# Autodesk Inventor assembly: поршень_шатун_палец
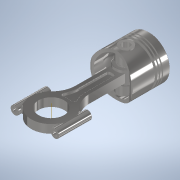
[picture p0: Inventor's stored thumbnail of the model, 180x180]
Saved by Autodesk Inventor 2021 (Build 250183000, 183)
## iProperties
Created: 2021-06-15
Part Number: поршень_шатун_палец
Document SubType Name: Assembly
Designer: panda
Author: panda
## Documents named in this file (4)
- C:\Users\panda\Desktop\vkrb\сборка\поршень_шатун_палец.iam
- C:\Users\panda\Desktop\vkrb\сборка\pin.ipt
- C:\Users\panda\Desktop\vkrb\сборка\piston.ipt
- C:\Users\panda\Desktop\vkrb\сборка\connecting_rod.ipt
## Components (3 placed, 3 different names)
1. pin:1 — Совмещение:2
2. piston:1 — Совмещение:1, Угол:1
3. connecting_rod:1 — Совмещение:1, Угол:1, Совмещение:2
## Relationships (3: Mate 2, Angle 1)
- Совмещение:1 [Mate]: piston:1 ↔ connecting_rod:1
- Угол:1 [Angle] (0 deg): piston:1 ↔ connecting_rod:1
- Совмещение:2 [Mate]: pin:1 ↔ connecting_rod:1
